# Autodesk Inventor assembly: edf_drone_v1
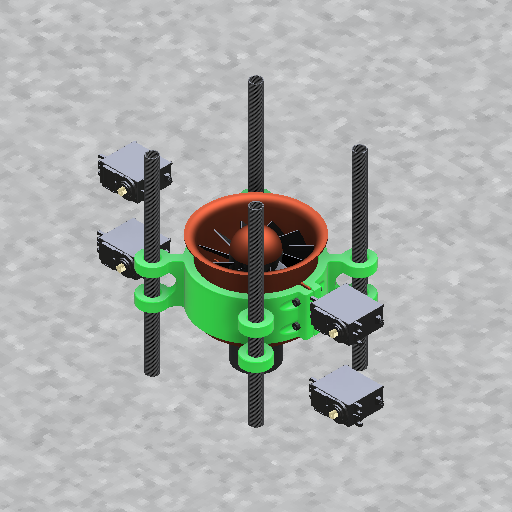
[picture p0: Inventor's stored thumbnail of the model, 512x512]
Saved by Autodesk Inventor 2026.2 (Build 302298010, 298A)
## iProperties
Created: 2026-03-12
Part Number: edf_drone_v1
Document SubType Name: Assembly
Designer: tngzj
Mass: 690.858 g
Surface Area: 1985.85 cm^2
Volume: 374.112 cm^3
Author: tngzj
## Documents named in this file (7)
- C:\Transformer-rl-retro-propulsion\CAD\EDF Drone v1\edf_drone_v1.iam
- C:\Transformer-rl-retro-propulsion\CAD\EDF Drone v1\Fan\fms 90mm edf.iam
- C:\Transformer-rl-retro-propulsion\CAD\EDF Drone v1\Structure\Carbon Fiber Tube 12mm x 10mm.ipt
- C:\Transformer-rl-retro-propulsion\CAD\EDF Drone v1\Structure\EDF Mount v1.ipt
- C:\Users\tngzj\OneDrive\Documents\Inventor\Content Center Files\R2026\en-US\ISO 14580_2011(E)\ISO 14580 M3.5x25-4.8.ipt
- C:\Users\tngzj\OneDrive\Documents\Inventor\Content Center Files\R2026\en-US\ISO 4032(2)\ISO 4032 - M3.5 - ISO.ipt
- C:\Transformer-rl-retro-propulsion\CAD\EDF Drone v1\Servo\MG996R Servo.ipt
## Components (19 placed, 6 different names)
1. fms 90mm edf:1 [sub-assembly] — Mate:10, Mate:11, Angle:3, Mate:13, Flush:2, Mate:14, Angle:4
2. EDF Mount v1:1 — Flush:2, Mate:14, Flush:3, Angle:4, Mate:19, Mate:20, Mate:21, Mate:23, Mate:24, Mate:25, Mate:27, Mate:28, Mate:31, Mate:32, Mate:33, Mate:35, Mate:36, Mate:37
3. EDF Mount v1:2 — Mate:13, Flush:3, Mate:22, Mate:26, Mate:29, Mate:30, Mate:34, Mate:38
4. Screw ISO 14580:2011(E) M3.5x25-4.8:2 — Mate:35, Mate:36
5. ISO 4032 M3.5:2 — Mate:37, Mate:38
6. Screw ISO 14580:2011(E) M3.5x25-4.8:3 — Mate:19, Mate:20
7. ISO 4032 M3.5:3 — Mate:21, Mate:22
8. Screw ISO 14580:2011(E) M3.5x25-4.8:4 — Mate:23, Mate:24
9. ISO 4032 M3.5:4 — Mate:25, Mate:26
10. Screw ISO 14580:2011(E) M3.5x25-4.8:5 — Mate:31, Mate:32
11. ISO 4032 M3.5:5 — Mate:33, Mate:34
12. Carbon Fiber Tube 12mm x 10mm:2 — Mate:28
13. Carbon Fiber Tube 12mm x 10mm:3 — Mate:29
14. Carbon Fiber Tube 12mm x 10mm:4 — Mate:30
15. Carbon Fiber Tube 12mm x 10mm:1 — Mate:27
16. MG996R Servo:1
17. MG996R Servo:2
18. MG996R Servo:3
19. MG996R Servo:4
## Relationships (28: Mate 24, Angle 2, Flush 2)
- Mate:10: fms 90mm edf:1
- Mate:11: fms 90mm edf:1
- Angle:3 (0 deg): fms 90mm edf:1
- Mate:13: fms 90mm edf:1 ↔ EDF Mount v1:2
- Flush:2: fms 90mm edf:1 ↔ EDF Mount v1:1
- Mate:14: fms 90mm edf:1 ↔ EDF Mount v1:1
- Flush:3: EDF Mount v1:1 ↔ EDF Mount v1:2
- Angle:4 (-180 deg): fms 90mm edf:1 ↔ EDF Mount v1:1
- Mate:19: EDF Mount v1:1 ↔ Screw ISO 14580:2011(E) M3.5x25-4.8:3
- Mate:20: EDF Mount v1:1 ↔ Screw ISO 14580:2011(E) M3.5x25-4.8:3
- Mate:21: EDF Mount v1:1 ↔ ISO 4032 M3.5:3
- Mate:22: EDF Mount v1:2 ↔ ISO 4032 M3.5:3
- Mate:23: EDF Mount v1:1 ↔ Screw ISO 14580:2011(E) M3.5x25-4.8:4
- Mate:24: EDF Mount v1:1 ↔ Screw ISO 14580:2011(E) M3.5x25-4.8:4
- Mate:25: EDF Mount v1:1 ↔ ISO 4032 M3.5:4
- Mate:26: EDF Mount v1:2 ↔ ISO 4032 M3.5:4
- Mate:27: EDF Mount v1:1 ↔ Carbon Fiber Tube 12mm x 10mm:1
- Mate:28: EDF Mount v1:1 ↔ Carbon Fiber Tube 12mm x 10mm:2
- Mate:29: EDF Mount v1:2 ↔ Carbon Fiber Tube 12mm x 10mm:3
- Mate:30: EDF Mount v1:2 ↔ Carbon Fiber Tube 12mm x 10mm:4
- Mate:31: EDF Mount v1:1 ↔ Screw ISO 14580:2011(E) M3.5x25-4.8:5
- Mate:32: EDF Mount v1:1 ↔ Screw ISO 14580:2011(E) M3.5x25-4.8:5
- Mate:33: EDF Mount v1:1 ↔ ISO 4032 M3.5:5
- Mate:34: EDF Mount v1:2 ↔ ISO 4032 M3.5:5
- Mate:35: EDF Mount v1:1 ↔ Screw ISO 14580:2011(E) M3.5x25-4.8:2
- Mate:36: EDF Mount v1:1 ↔ Screw ISO 14580:2011(E) M3.5x25-4.8:2
- Mate:37: EDF Mount v1:1 ↔ ISO 4032 M3.5:2
- Mate:38: EDF Mount v1:2 ↔ ISO 4032 M3.5:2
